# Autodesk Inventor assembly: stojak
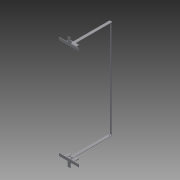
[picture p0: Inventor's stored thumbnail of the model, 180x180]
Saved by Autodesk Inventor 2014 (Build 180170000, 170)
## iProperties
Created: 2014-12-22
Part Number: stojak
Document SubType Name: Assembly
Designer: Kuba
Author: Kuba
## Documents named in this file (11)
- C:\Users\Kuba\Dysk Google\synergia\RoboDrift2015\Pomiar czasu\konstrukcja\stojak.iam
- C:\Users\Kuba\Dysk Google\synergia\RoboDrift2015\Pomiar czasu\konstrukcja\podstawa d.ipt
- C:\Users\Kuba\Dysk Google\synergia\RoboDrift2015\Pomiar czasu\konstrukcja\czujnik.ipt
- C:\Users\Kuba\Dysk Google\synergia\RoboDrift2015\Pomiar czasu\konstrukcja\podstawa krótka.ipt
- C:\Users\Kuba\Dysk Google\synergia\RoboDrift2015\Pomiar czasu\konstrukcja\płaskownik.ipt
- C:\Users\Kuba\Documents\Inventor\Content Center Files\R2014\pl-PL\ISO 7050 - C-Z(1)\ISO 7050 - ST4,8 x 9,5 - C - ZDIN ISO.ipt
- C:\Users\Kuba\Dysk Google\synergia\RoboDrift2015\Pomiar czasu\konstrukcja\DIN EN 10056-1 - L60x60x5-40.ipt
- C:\Users\Kuba\Dysk Google\synergia\RoboDrift2015\Pomiar czasu\konstrukcja\deska300x80.ipt
- C:\Users\Kuba\Dysk Google\synergia\RoboDrift2015\Pomiar czasu\konstrukcja\deska120x80.ipt
- C:\Users\Kuba\Dysk Google\synergia\RoboDrift2015\Pomiar czasu\konstrukcja\listwa20x20x50.ipt
- C:\Users\Kuba\Dysk Google\synergia\RoboDrift2015\Pomiar czasu\konstrukcja\przęsło.ipt
## Components (41 placed, 11 different names)
1. podstawa d:1 — Zestawiający:1, Zestawiający:2, Równoległy:1, Równoległy:2, Zestawiający:3, Zestawiający:4, Zestawiający:5, Zestawiający:6, Równoległy:5, Zestawiający:8, Równoległy:9, Zestawiający:10, Zestawiający:15, Równoległy:15, Równoległy:16, Zestawiający:16, Równoległy:35, Równoległy:36
2. czujnik:1 — Równoległy:2, Zestawiający:3, Równoległy:4, Zestawiający:17, Zestawiający:18, Zestawiający:20
3. deska 150x80 — Zestawiający:1, Zestawiający:2, Równoległy:1, Równoległy:3, Równoległy:4, Zestawiający:12, Zestawiający:14, Zestawiający:19, Równoległy:17, Zestawiający:42
4. płaskownik:1 — Zestawiający:4, Zestawiający:5, Równoległy:3, Wstaw:1, Wstaw:2, Wstaw:3, Wstaw:4, Wstaw:5, Wstaw:6
5. DIN ISO 7050 - C-Z ST4,8 x 9,5 - C - Z:1 — Wstaw:1
6. DIN ISO 7050 - C-Z ST4,8 x 9,5 - C - Z:2 — Wstaw:2
7. DIN ISO 7050 - C-Z ST4,8 x 9,5 - C - Z:3 — Wstaw:3
8. DIN ISO 7050 - C-Z ST4,8 x 9,5 - C - Z:4 — Wstaw:4
9. DIN ISO 7050 - C-Z ST4,8 x 9,5 - C - Z:5 — Wstaw:6
10. DIN ISO 7050 - C-Z ST4,8 x 9,5 - C - Z:6 — Wstaw:5
11. DIN EN 10056-1 - L60x60x5-40:1 — Zestawiający:6, Równoległy:5, Zestawiający:7, Równoległy:6
12. podstawa krótka:2 — Zestawiający:7, Zestawiający:8, Równoległy:6, Zestawiający:11, Równoległy:11, Równoległy:12
13. DIN EN 10056-1 - L60x60x5-40:2 — Równoległy:8, Zestawiający:10
14. podstawa krótka:3 — Równoległy:8, Równoległy:9, Równoległy:10
15. deska300x80:1 — Zestawiający:11, Równoległy:10, Równoległy:11, Równoległy:12, Zestawiający:12, Równoległy:14, Zestawiający:13
16. deska120x80:1 — Równoległy:14, Zestawiający:13, Zestawiający:14, Zestawiający:41, Równoległy:34, Zestawiający:46
17. listwa20x20x50:1 — Zestawiający:15, Równoległy:15, Zestawiający:18
18. listwa20x20x50:2 — Równoległy:16, Zestawiający:16, Zestawiający:17
19. listwa20x20x50:3 — Zestawiający:19, Zestawiający:20, Równoległy:17
20. podstawa d:2 — Równoległy:36
21. czujnik:2
22. podstawa krótka:4 — Równoległy:35
23. płaskownik:2
24. DIN ISO 7050 - C-Z ST4,8 x 9,5 - C - Z:7
25. DIN ISO 7050 - C-Z ST4,8 x 9,5 - C - Z:8
26. DIN ISO 7050 - C-Z ST4,8 x 9,5 - C - Z:9
27. DIN ISO 7050 - C-Z ST4,8 x 9,5 - C - Z:10
28. DIN ISO 7050 - C-Z ST4,8 x 9,5 - C - Z:11
29. DIN ISO 7050 - C-Z ST4,8 x 9,5 - C - Z:12
30. DIN EN 10056-1 - L60x60x5-40:3
31. podstawa krótka:5
32. DIN EN 10056-1 - L60x60x5-40:4
33. podstawa krótka:6
34. deska300x80:2
35. deska120x80:2 — Równoległy:43, Zestawiający:43
36. listwa20x20x50:4
37. listwa20x20x50:5
38. listwa20x20x50:6
39. przęsło:1 — Zestawiający:41, Równoległy:34, Równoległy:43, Zestawiający:42, Zestawiający:44, Równoległy:44, Zestawiający:45, Równoległy:45
40. DIN EN 10056-1 - L60x60x5-40:5 — Zestawiający:43, Zestawiający:44, Równoległy:44
41. DIN EN 10056-1 - L60x60x5-40:6 — Zestawiający:45, Zestawiający:46, Równoległy:45
## Relationships (96: Mate 46, Flush 38, Insert 12)
- Zestawiający:1 [Mate]: podstawa d:1 ↔ deska 150x80
- Zestawiający:2 [Mate]: podstawa d:1 ↔ deska 150x80
- Równoległy:1 [Flush]: podstawa d:1 ↔ deska 150x80
- Równoległy:2 [Flush]: podstawa d:1 ↔ czujnik:1
- Zestawiający:3 [Mate]: podstawa d:1 ↔ czujnik:1
- Zestawiający:4 [Mate]: podstawa d:1 ↔ płaskownik:1
- Zestawiający:5 [Mate]: podstawa d:1 ↔ płaskownik:1
- Równoległy:3 [Flush]: deska 150x80 ↔ płaskownik:1
- Wstaw:1 [Insert] (-4.65 mm): płaskownik:1 ↔ DIN ISO 7050 - C-Z ST4,8 x 9,5 - C - Z:1
- Wstaw:2 [Insert] (-2.25 mm): płaskownik:1 ↔ DIN ISO 7050 - C-Z ST4,8 x 9,5 - C - Z:2
- Wstaw:3 [Insert] (-2.25 mm): płaskownik:1 ↔ DIN ISO 7050 - C-Z ST4,8 x 9,5 - C - Z:3
- Wstaw:4 [Insert] (-4.65 mm): płaskownik:1 ↔ DIN ISO 7050 - C-Z ST4,8 x 9,5 - C - Z:4
- Wstaw:5 [Insert] (-2.25 mm): płaskownik:1 ↔ DIN ISO 7050 - C-Z ST4,8 x 9,5 - C - Z:6
- Wstaw:6 [Insert] (-4.65 mm): płaskownik:1 ↔ DIN ISO 7050 - C-Z ST4,8 x 9,5 - C - Z:5
- Równoległy:4 [Flush]: czujnik:1 ↔ deska 150x80
- Zestawiający:6 [Mate]: podstawa d:1 ↔ DIN EN 10056-1 - L60x60x5-40:1
- Równoległy:5 [Flush] (10 mm): podstawa d:1 ↔ DIN EN 10056-1 - L60x60x5-40:1
- Zestawiający:7 [Mate]: DIN EN 10056-1 - L60x60x5-40:1 ↔ podstawa krótka:2
- Zestawiający:8 [Mate]: podstawa d:1 ↔ podstawa krótka:2
- Równoległy:6 [Flush] (20 mm): DIN EN 10056-1 - L60x60x5-40:1 ↔ podstawa krótka:2
- [Mate]: DIN EN 10056-1 - L60x60x5-40:2 ↔ podstawa krótka:3
- [Flush] (20 mm): DIN EN 10056-1 - L60x60x5-40:2 ↔ podstawa krótka:3
- Równoległy:8 [Flush]: DIN EN 10056-1 - L60x60x5-40:2 ↔ podstawa krótka:3
- Równoległy:9 [Flush]: podstawa d:1 ↔ podstawa krótka:3
- Zestawiający:10 [Mate]: podstawa d:1 ↔ DIN EN 10056-1 - L60x60x5-40:2
- Zestawiający:11 [Mate]: podstawa krótka:2 ↔ deska300x80:1
- Równoległy:10 [Flush]: podstawa krótka:3 ↔ deska300x80:1
- Równoległy:11 [Flush]: podstawa krótka:2 ↔ deska300x80:1
- Równoległy:12 [Flush]: podstawa krótka:2 ↔ deska300x80:1
- Zestawiający:12 [Mate]: deska 150x80 ↔ deska300x80:1
- Równoległy:14 [Flush]: deska300x80:1 ↔ deska120x80:1
- Zestawiający:13 [Mate]: deska300x80:1 ↔ deska120x80:1
- Zestawiający:14 [Mate]: deska 150x80 ↔ deska120x80:1
- Zestawiający:15 [Mate]: podstawa d:1 ↔ listwa20x20x50:1
- Równoległy:15 [Flush] (15 mm): podstawa d:1 ↔ listwa20x20x50:1
- Równoległy:16 [Flush] (15 mm): podstawa d:1 ↔ listwa20x20x50:2
- Zestawiający:16 [Mate]: podstawa d:1 ↔ listwa20x20x50:2
- Zestawiający:17 [Mate]: czujnik:1 ↔ listwa20x20x50:2
- Zestawiający:18 [Mate]: czujnik:1 ↔ listwa20x20x50:1
- Zestawiający:19 [Mate]: deska 150x80 ↔ listwa20x20x50:3
- Zestawiający:20 [Mate]: czujnik:1 ↔ listwa20x20x50:3
- Równoległy:17 [Flush]: deska 150x80 ↔ listwa20x20x50:3
- [Mate]: podstawa d:2 ↔ podstawa krótka:4
- [Mate]: podstawa d:2 ↔ podstawa krótka:4
- [Flush]: podstawa d:2 ↔ podstawa krótka:4
- [Flush]: podstawa d:2 ↔ czujnik:2
- [Mate]: podstawa d:2 ↔ czujnik:2
- [Mate]: podstawa d:2 ↔ płaskownik:2
- [Mate]: podstawa d:2 ↔ płaskownik:2
- [Flush]: podstawa krótka:4 ↔ płaskownik:2
- [Insert] (-4.65 mm): płaskownik:2 ↔ DIN ISO 7050 - C-Z ST4,8 x 9,5 - C - Z:7
- [Insert] (-2.25 mm): płaskownik:2 ↔ DIN ISO 7050 - C-Z ST4,8 x 9,5 - C - Z:8
- [Insert] (-2.25 mm): płaskownik:2 ↔ DIN ISO 7050 - C-Z ST4,8 x 9,5 - C - Z:9
- [Insert] (-4.65 mm): płaskownik:2 ↔ DIN ISO 7050 - C-Z ST4,8 x 9,5 - C - Z:10
- [Insert] (-2.25 mm): płaskownik:2 ↔ DIN ISO 7050 - C-Z ST4,8 x 9,5 - C - Z:12
- [Insert] (-4.65 mm): płaskownik:2 ↔ DIN ISO 7050 - C-Z ST4,8 x 9,5 - C - Z:11
- [Flush]: czujnik:2 ↔ podstawa krótka:4
- [Mate]: podstawa d:2 ↔ DIN EN 10056-1 - L60x60x5-40:3
- [Flush] (10 mm): podstawa d:2 ↔ DIN EN 10056-1 - L60x60x5-40:3
- [Mate]: DIN EN 10056-1 - L60x60x5-40:3 ↔ podstawa krótka:5
- [Mate]: podstawa d:2 ↔ podstawa krótka:5
- [Flush] (20 mm): DIN EN 10056-1 - L60x60x5-40:3 ↔ podstawa krótka:5
- [Mate]: DIN EN 10056-1 - L60x60x5-40:4 ↔ podstawa krótka:6
- [Flush] (20 mm): DIN EN 10056-1 - L60x60x5-40:4 ↔ podstawa krótka:6
- [Flush]: DIN EN 10056-1 - L60x60x5-40:4 ↔ podstawa krótka:6
- [Flush]: podstawa d:2 ↔ podstawa krótka:6
- [Mate]: podstawa d:2 ↔ DIN EN 10056-1 - L60x60x5-40:4
- [Mate]: podstawa krótka:5 ↔ deska300x80:2
- [Flush]: podstawa krótka:6 ↔ deska300x80:2
- [Flush]: podstawa krótka:5 ↔ deska300x80:2
- [Flush]: podstawa krótka:5 ↔ deska300x80:2
- [Mate]: podstawa krótka:4 ↔ deska300x80:2
- [Flush]: deska300x80:2 ↔ deska120x80:2
- [Mate]: deska300x80:2 ↔ deska120x80:2
- [Mate]: podstawa krótka:4 ↔ deska120x80:2
- [Mate]: podstawa d:2 ↔ listwa20x20x50:4
- [Flush] (15 mm): podstawa d:2 ↔ listwa20x20x50:4
- [Flush] (15 mm): podstawa d:2 ↔ listwa20x20x50:5
- [Mate]: podstawa d:2 ↔ listwa20x20x50:5
- [Mate]: czujnik:2 ↔ listwa20x20x50:5
- [Mate]: czujnik:2 ↔ listwa20x20x50:4
- [Mate]: podstawa krótka:4 ↔ listwa20x20x50:6
- [Mate]: czujnik:2 ↔ listwa20x20x50:6
- [Flush]: podstawa krótka:4 ↔ listwa20x20x50:6
- Zestawiający:41 [Mate]: deska120x80:1 ↔ przęsło:1
- Równoległy:34 [Flush]: deska120x80:1 ↔ przęsło:1
- Równoległy:43 [Flush]: deska120x80:2 ↔ przęsło:1
- Równoległy:35 [Flush]: podstawa d:1 ↔ podstawa krótka:4
- Równoległy:36 [Flush]: podstawa d:1 ↔ podstawa d:2
- Zestawiający:42 [Mate]: deska 150x80 ↔ przęsło:1
- Zestawiający:43 [Mate]: deska120x80:2 ↔ DIN EN 10056-1 - L60x60x5-40:5
- Zestawiający:44 [Mate]: przęsło:1 ↔ DIN EN 10056-1 - L60x60x5-40:5
- Równoległy:44 [Flush]: przęsło:1 ↔ DIN EN 10056-1 - L60x60x5-40:5
- Zestawiający:45 [Mate]: przęsło:1 ↔ DIN EN 10056-1 - L60x60x5-40:6
- Zestawiający:46 [Mate]: deska120x80:1 ↔ DIN EN 10056-1 - L60x60x5-40:6
- Równoległy:45 [Flush]: przęsło:1 ↔ DIN EN 10056-1 - L60x60x5-40:6
## Named parameters: d25_d22 = 0 mm, d26_d24 = 20 mm, d47_d36 = 0 mm, d48_d37 = 0 mm, d49_d38 = 0 mm, d50_d39 = 15 mm, d51_d40 = 15 mm, d52_d41 = 0 mm, d53_d42 = 0 mm, d54_d43 = 0 mm, d55_d44 = 0 mm, d56_d17 = -2.25 mm, d57_d18 = -4.65 mm, d58_d19 = 0 mm, d59_d20 = 0 mm, d60_d21 = 10 mm, d61_d22 = 0 mm, d62_d23 = 0 mm, d63_d13 = -2.25 mm, d64_d15 = -2.25 mm, d65_d16 = -4.65 mm, d66_d45 = 0 mm, d67_d46 = 0 mm, d68_d24 = 20 mm, d69_d25_d22 = 0 mm, d70_d26_d24 = 20 mm, d71_d27 = 0 mm, d72_d28 = 0 mm, d73_d29 = 0 mm, d74_d30 = 0 mm, d75_d31 = 0 mm, d76_d32 = 0 mm, d77_d33 = 0 mm, d78_d34 = 0 mm, d79_d35 = 0 mm, d80_d3 = 0 mm, d81_d4 = 0 mm, d82_d5 = 0 mm, d83_d7 = 0 mm, d84_d8 = 0 mm, d85_d12 = -4.65 mm, d86_d0 = 0 mm, d87_d1 = 0 mm, d88_d2 = 0 mm
